# Autodesk Inventor assembly: Shock_Absorber_MIR
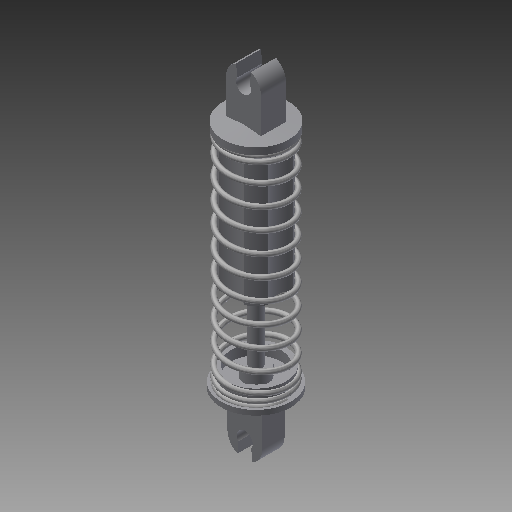
[picture p0: Inventor's stored thumbnail of the model, 512x512]
Saved by Autodesk Inventor 2019 (Build 230136000, 136)
## iProperties
Created: 2019-03-03
Part Number: Shock_Absorber_MIR
Document SubType Name: Assembly
Designer: alarr
Author: alarr
## Documents named in this file (4)
- C:\Users\alarr\OneDrive\Documents\Inventor\Mr.Green\Shock_Absorber_MIR.iam
- C:\Users\alarr\OneDrive\Documents\Inventor\Mr.Green\Bottom_MIR.ipt
- C:\Users\alarr\OneDrive\Documents\Inventor\Mr.Green\Top_MIR.ipt
- C:\Users\alarr\OneDrive\Documents\Inventor\Mr.Green\Shock_Absorber\Design Accelerator\Compress Spring2_MIR.iam
## Components (3 placed, 3 different names)
1. Bottom_MIR:1 — Angle:1, Mate:1, Flush:1
2. Top_MIR:1 — Angle:1, Mate:1, Mate:4
3. Compress Spring2_MIR:1 [sub-assembly] — Mate:4, Flush:1, Mate:3
## Relationships (5: Mate 4, Angle 1)
- Angle:1 (0 deg): Bottom_MIR:1 ↔ Top_MIR:1
- Mate:1: Bottom_MIR:1 ↔ Top_MIR:1
- Mate:4: Top_MIR:1 ↔ Compress Spring2_MIR:1
- Flush:1 [Mate]: Bottom_MIR:1 ↔ Compress Spring2_MIR:1
- Mate:3: Compress Spring2_MIR:1
